# Autodesk Inventor assembly: Assembly-PCB alone
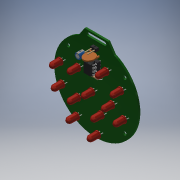
[picture p0: Inventor's stored thumbnail of the model, 180x180]
Saved by Autodesk Inventor 2018.3 (Build 223284000, 284)
## iProperties
Company: UNH Makerspace
Created: 2019-07-21
Part Number: Assembly-PCB alone
Document SubType Name: Assembly
Designer: Electro707
Engineer: Jamal Bouajjaj
Author: Electro707
Title: Blinking Ornament
Revision Number: N/A
## iProperties of the stored document LED_D5.0mm.iam
Created: 2019-07-21
Part Number: LED_D5.0mm
Document SubType Name: Assembly
Designer: Electro707
Author: Electro707
## iProperties of the stored document SOLID_4.ipt
Created: 2019-07-21
Part Number: SOLID_4
Material: Generic
Document SubType Name: Modeling
Designer: Electro707
Density: 1 g/cm^3
Appearance: Default
Author: Electro707
## iProperties of the stored document R_1206_3216Metric.iam
Created: 2019-11-21
Part Number: R_1206_3216Metric
Document SubType Name: Assembly
Designer: Electro707
Author: Electro707
## iProperties of the stored document SOLID_5.ipt
Created: 2019-07-21
Part Number: SOLID_5
Material: Generic
Document SubType Name: Modeling
Designer: Electro707
Density: 1 g/cm^3
Appearance: Default
Author: Electro707
## iProperties of the stored document PCB.iam
Created: 2019-12-21
Part Number: PCB
Description: KiCad electronic assembly
Document SubType Name: Assembly
Designer: Electro707
Authority: Unknown
Company: A Company
Sending System: KiCad to STEP converter
Preprocessor: Open CASCADE STEP processor 6.9
Title: PCB.step
Author: An Author
## iProperties of the stored document PinHeader_1x02_P2.54mm_Vertical.iam
Created: 2019-07-21
Part Number: PinHeader_1x02_P2.54mm_Vertical
Document SubType Name: Assembly
Designer: Electro707
Author: Electro707
## iProperties of the stored document SOLID_3.ipt
Created: 2019-07-21
Part Number: SOLID_3
Material: Generic
Document SubType Name: Modeling
Designer: Electro707
Density: 1 g/cm^3
Appearance: Default
Author: Electro707
## iProperties of the stored document SOLID.ipt
Created: 2019-11-21
Part Number: SOLID
Material: Generic
Document SubType Name: Modeling
Designer: Electro707
Density: 1 g/cm^3
Appearance: Default
Author: Electro707
## iProperties of the stored document SOLID_2.ipt
Created: 2019-07-21
Part Number: SOLID_2
Material: Generic
Document SubType Name: Modeling
Designer: Electro707
Density: 1 g/cm^3
Appearance: Default
Author: Electro707
## iProperties of the stored document Fuse_BelFuse_0ZRE_0ZRE0005FF_L8.3mm_W3.8mm.iam
Created: 2019-12-22
Part Number: Fuse_BelFuse_0ZRE_0ZRE0005FF_L8.3mm_W3.8mm
Document SubType Name: Assembly
Designer: Jamal Bouajjaj
Author: Jamal Bouajjaj
## iProperties of the stored document SOLID_1.ipt
Created: 2019-07-21
Part Number: SOLID_1
Material: Generic
Document SubType Name: Modeling
Designer: Electro707
Density: 1 g/cm^3
Appearance: Default
Author: Electro707
## iProperties of the stored document C_1206_3216Metric.iam
Created: 2019-11-21
Part Number: C_1206_3216Metric
Document SubType Name: Assembly
Designer: Electro707
Author: Electro707
## iProperties of the stored document CP_Radial_D5.0mm_P2.50mm.iam
Created: 2019-07-21
Part Number: CP_Radial_D5.0mm_P2.50mm
Document SubType Name: Assembly
Designer: Electro707
Author: Electro707
## iProperties of the stored document SOLID.ipt
Created: 2019-07-21
Part Number: SOLID
Material: Generic
Document SubType Name: Modeling
Designer: Electro707
Density: 1 g/cm^3
Appearance: Default
Author: Electro707
## iProperties of the stored document R_Axial_DIN0207_L6.3mm_D2.5mm_P10.16mm_Horizontal.iam
Created: 2019-07-21
Part Number: R_Axial_DIN0207_L6.3mm_D2.5mm_P10.16mm_Horizontal
Document SubType Name: Assembly
Designer: Electro707
Author: Electro707
## iProperties of the stored document DIP-8_W7.62mm_Socket.iam
Created: 2019-07-21
Part Number: DIP-8_W7.62mm_Socket
Document SubType Name: Assembly
Designer: Electro707
Author: Electro707
## iProperties of the stored document COMPOUND.ipt
Created: 2019-07-21
Part Number: COMPOUND
Material: Generic
Document SubType Name: Modeling
Designer: Electro707
Density: 1 g/cm^3
Appearance: Default
Author: Electro707
## iProperties of the stored document SOLID.ipt
Created: 2019-12-22
Part Number: SOLID
Material: Generic
Document SubType Name: Modeling
Designer: Jamal Bouajjaj
Density: 1 g/cm^3
Appearance: Default
Author: Jamal Bouajjaj
## Documents named in this file (21)
- **F:\Projects\UNH MakerSpace Kits\2019 - Winter Holiday\Ornament\CAD-Inventor\Assembly-PCB alone.iam*LocalDocs*xEonbvse52mauusw4Iqhc32puUc*LED_D5.0mm.iam
- **F:\Projects\UNH MakerSpace Kits\2019 - Winter Holiday\Ornament\CAD-Inventor\Assembly-PCB alone.iam*LocalDocs*xAtyid1pnBbzwecgtBvikhpk5Th*SOLID_3.ipt
- **F:\Projects\UNH MakerSpace Kits\2019 - Winter Holiday\Ornament\CAD-Inventor\Assembly-PCB alone.iam*LocalDocs*xAl2hsrkzC4rouboz3pj2mzgpRg*SOLID_4.ipt
- **F:\Projects\UNH MakerSpace Kits\2019 - Winter Holiday\Ornament\CAD-Inventor\Assembly-PCB alone.iam*LocalDocs*x2qmq03u33xhbuvs1DzkndkbtJa*R_1206_3216Metric.iam
- **F:\Projects\UNH MakerSpace Kits\2019 - Winter Holiday\Ornament\CAD-Inventor\Assembly-PCB alone.iam*LocalDocs*xQhtn1zva24ksevkcNdtxirvdUe*SOLID_2.ipt
- **F:\Projects\UNH MakerSpace Kits\2019 - Winter Holiday\Ornament\CAD-Inventor\Assembly-PCB alone.iam*LocalDocs*x1dnbwgowLuskex00Tdg04ttlUh*SOLID_5.ipt
- **F:\Projects\UNH MakerSpace Kits\2019 - Winter Holiday\Ornament\CAD-Inventor\Assembly-PCB alone.iam*LocalDocs*x5n2ylh3rTo2rez4w0knx3dshBg*PCB.iam
- **F:\Projects\UNH MakerSpace Kits\2019 - Winter Holiday\Ornament\CAD-Inventor\Assembly-PCB alone.iam*LocalDocs*xZhqa0hjb0wmwuc4uDdkpbvgzDf*R_Axial_DIN0207_L6.3mm_D2.5mm_P10.16mm_Horizontal.iam
- **F:\Projects\UNH MakerSpace Kits\2019 - Winter Holiday\Ornament\CAD-Inventor\Assembly-PCB alone.iam*LocalDocs*xChft5v0fLjxzedgaJnpc3qrkHe*PinHeader_1x02_P2.54mm_Vertical.iam
- **F:\Projects\UNH MakerSpace Kits\2019 - Winter Holiday\Ornament\CAD-Inventor\Assembly-PCB alone.iam*LocalDocs*xVzta3gnxT0tpu0om5ealklsjCf*DIP-8_W7.62mm_Socket.iam
- **F:\Projects\UNH MakerSpace Kits\2019 - Winter Holiday\Ornament\CAD-Inventor\Assembly-PCB alone.iam*LocalDocs*xUrplyq5jCdomeawbXkayqukrEd*CP_Radial_D5.0mm_P2.50mm.iam
- **F:\Projects\UNH MakerSpace Kits\2019 - Winter Holiday\Ornament\CAD-Inventor\Assembly-PCB alone.iam*LocalDocs*xZswqba0yM1scuxkn4c1z0l1lEh*COMPOUND.ipt
- **F:\Projects\UNH MakerSpace Kits\2019 - Winter Holiday\Ornament\CAD-Inventor\Assembly-PCB alone.iam*LocalDocs*xOt044fp2FnifemgaIsuivd5z5g*C_1206_3216Metric.iam
- **F:\Projects\UNH MakerSpace Kits\2019 - Winter Holiday\Ornament\CAD-Inventor\Assembly-PCB alone.iam*LocalDocs*xOpucott4Nyzfuh0gOtksof2iNd*Fuse_BelFuse_0ZRE_0ZRE0005FF_L8.3mm_W3.8mm.iam
- **F:\Projects\UNH MakerSpace Kits\2019 - Winter Holiday\Ornament\CAD-Inventor\Assembly-PCB alone.iam*LocalDocs*xCxcuxpinKjj0esorTfdgldvpRf*SOLID.ipt
- **F:\Projects\UNH MakerSpace Kits\2019 - Winter Holiday\Ornament\CAD-Inventor\Assembly-PCB alone.iam*LocalDocs*xUbianyycD4etuyosG1m31ujuGg*SOLID.ipt
- **F:\Projects\UNH MakerSpace Kits\2019 - Winter Holiday\Ornament\CAD-Inventor\Assembly-PCB alone.iam*LocalDocs*xNibf0b5440nvuzk2QzfsvprwGf*SOLID_1.ipt
- **F:\Projects\UNH MakerSpace Kits\2019 - Winter Holiday\Ornament\CAD-Inventor\Assembly-PCB alone.iam*LocalDocs*xZv0zn2z3Xmmae24pC25sskwr2d*SOLID.ipt
- F:\Projects\UNH MakerSpace Kits\2019 - Winter Holiday\Ornament\CAD-Inventor\Assembly-PCB alone.iam
- F:\Kicad\3d Models\DIP-8_W7.62mm.ipt
- F:\Projects\UNH MakerSpace Kits\2019 - Winter Holiday\Ornament\PCB\PCB.step
## Components (2 placed, 2 different names)
1. PCB:1 [sub-assembly] — Cylindrical:1, Cylindrical:2, Mate:1
2. DIP-8_W7.62mm:1 — Cylindrical:1, Cylindrical:2, Mate:1
## Relationships (3: CylindricalJoint 2, Mate 1)
- Cylindrical:1: PCB:1 ↔ DIP-8_W7.62mm:1
- Cylindrical:2: PCB:1 ↔ DIP-8_W7.62mm:1
- Mate:1: PCB:1 ↔ DIP-8_W7.62mm:1
